# Autodesk Inventor assembly: Binary Clock
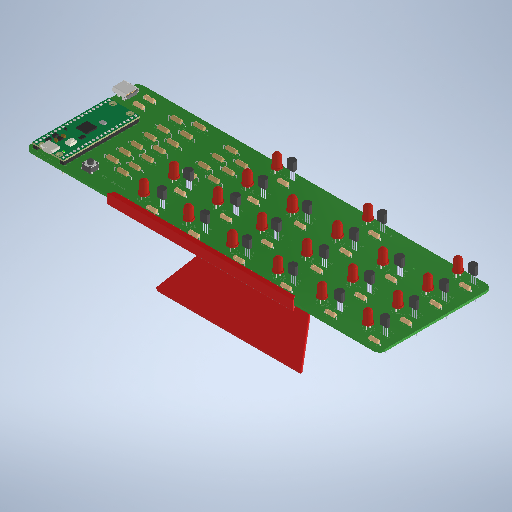
[picture p0: Inventor's stored thumbnail of the model, 512x512]
Saved by Autodesk Inventor 2025.3 (Build 293356000, 356)
## iProperties
Company: Kicad
Created: 2025-11-09
Part Number: Binary Clock
Description: KiCad electronic assembly
Document SubType Name: Assembly
Designer: User
Authority: Unknown
Sending System: KiCad to STEP converter
Preprocessor: Open CASCADE STEP processor 7.9
Title: Binary Clock.step
Author: Pcbnew
## Documents named in this file (11)
- C:\Users\User\Documents\KiCad\Binary Clock\Binary Clock\Binary Clock\Binary Clock\Binary Clock.iam
- C:\Users\User\Documents\KiCad\Binary Clock\Binary Clock\Binary Clock\Binary Clock\LED_D5.0mm.ipt
- C:\Users\User\Documents\KiCad\Binary Clock\Binary Clock\Binary Clock\Binary Clock\R_Axial_DIN0207_L6.3mm_D2.5mm_P7.62mm_Horizontal.ipt
- C:\Users\User\Documents\KiCad\Binary Clock\Binary Clock\Binary Clock\Binary Clock\RaspberryPi_Pico_H.iam
- C:\Users\User\Documents\KiCad\Binary Clock\Binary Clock\Binary Clock\Binary Clock\Binary Clock_silkscreen.ipt
- C:\Users\User\Documents\KiCad\Binary Clock\Binary Clock\Binary Clock\Binary Clock\Binary Clock_PCB.ipt
- C:\Users\User\3D\PC Case\Part14.ipt
- C:\Users\User\Documents\KiCad\Binary Clock\Binary Clock\Binary Clock\Binary Clock\R1.ipt
- C:\Users\User\Documents\KiCad\Binary Clock\Binary Clock\Binary Clock\Binary Clock\Same_Sky_TS02-66-70-BK-160-LCR-D.ipt
- C:\Users\User\Documents\KiCad\Binary Clock\Binary Clock\Binary Clock\Binary Clock\usb4085-gf-a.iam
- C:\Users\User\Downloads\BC547BBU\BC547BBU\BC547BBU.iam
## Components (88 placed, 50 different names)
1. 1
2. 2
3. 3
4. 4
5. 5
6. 6
7. 7
8. 8
9. 9
10. 10
11. 11
12. 12
13. 13
14. 14
15. 15
16. 16
17. 17
18. 18
19. 19
20. 20
21. 21
22. 22
23. 23
24. 24
25. 25
26. 26
27. 27
28. 28
29. 29
30. 30
31. 31
32. 32
33. 33
34. 34
35. 35
36. 36
37. 39 [sub-assembly]
38. 40
39. 41
40. 42
41. 43
42. 44
43. 45
44. 46
45. 47 — Flush:1, Mate:1, Mate:2, Mate:3, Mate:4, Mate:5, Mate:6, Mate:7, Mate:8, Mate:9, Mate:10, Mate:11, Mate:12, Mate:13, Mate:14, Mate:15, Mate:16, Mate:17, Mate:18, Mate:19, Mate:20, Mate:21, Mate:22, Mate:23, Mate:24, Mate:25, Mate:26, Mate:27, Mate:28, Mate:29, Mate:30, Mate:31, Mate:32, Mate:33, Mate:34, Mate:35, Mate:36, Mate:37, Mate:38, Mate:39, Mate:40, Mate:41, Mate:42
46. Part14:1 — Flush:1
47. R1:1 — Mate:2
48. R1:2 — Mate:1
49. R1:4 — Mate:3
50. R1:5 — Mate:6
51. R1:6 — Mate:4
52. R1:7 — Mate:12
53. R1:8 — Mate:8
54. R1:9 — Mate:7
55. R1:10 — Mate:5
56. R1:11 — Mate:15
57. R1:12 — Mate:14
58. R1:13 — Mate:9
59. R1:14 — Mate:11
60. R1:15 — Mate:18
61. R1:18 — Mate:17
62. R1:20 — Mate:20
63. R1:21 — Mate:13
64. R1:22 — Mate:19
65. R1:24 — Mate:16
66. R1:25 — Mate:10
67. Same_Sky_TS02-66-70-BK-160-LCR-D:1 — Mate:21
68. usb4085-gf-a:1 [sub-assembly] — Mate:22
69. BC547BBU:1 [sub-assembly] — Mate:23
70. BC547BBU:2 [sub-assembly] — Mate:24
71. BC547BBU:3 [sub-assembly] — Mate:25
72. BC547BBU:4 [sub-assembly] — Mate:26
73. BC547BBU:5 [sub-assembly] — Mate:33
74. BC547BBU:6 [sub-assembly] — Mate:27
75. BC547BBU:7 [sub-assembly] — Mate:28
76. BC547BBU:8 [sub-assembly] — Mate:32
77. BC547BBU:9 [sub-assembly] — Mate:31
78. BC547BBU:10 [sub-assembly] — Mate:29
79. BC547BBU:11 [sub-assembly] — Mate:30
80. BC547BBU:12 [sub-assembly] — Mate:37
81. BC547BBU:13 [sub-assembly] — Mate:35
82. BC547BBU:14 [sub-assembly] — Mate:34
83. BC547BBU:15 [sub-assembly] — Mate:38
84. BC547BBU:16 [sub-assembly] — Mate:36
85. BC547BBU:17 [sub-assembly] — Mate:40
86. BC547BBU:18 [sub-assembly] — Mate:42
87. BC547BBU:19 [sub-assembly] — Mate:39
88. BC547BBU:20 [sub-assembly] — Mate:41
## Relationships (43: Mate 42, Flush 1)
- Flush:1: 47 ↔ Part14:1
- Mate:1: 47 ↔ R1:2
- Mate:2: 47 ↔ R1:1
- Mate:3: 47 ↔ R1:4
- Mate:4: 47 ↔ R1:6
- Mate:5: 47 ↔ R1:10
- Mate:6: 47 ↔ R1:5
- Mate:7: 47 ↔ R1:9
- Mate:8: 47 ↔ R1:8
- Mate:9: 47 ↔ R1:13
- Mate:10: 47 ↔ R1:25
- Mate:11: 47 ↔ R1:14
- Mate:12: 47 ↔ R1:7
- Mate:13: 47 ↔ R1:21
- Mate:14: 47 ↔ R1:12
- Mate:15: 47 ↔ R1:11
- Mate:16: 47 ↔ R1:24
- Mate:17: 47 ↔ R1:18
- Mate:18: 47 ↔ R1:15
- Mate:19: 47 ↔ R1:22
- Mate:20: 47 ↔ R1:20
- Mate:21: 47 ↔ Same_Sky_TS02-66-70-BK-160-LCR-D:1
- Mate:22 (0.05 mm): 47 ↔ usb4085-gf-a:1
- Mate:23 (6 mm): 47 ↔ BC547BBU:1
- Mate:24 (6 mm): 47 ↔ BC547BBU:2
- Mate:25 (6 mm): 47 ↔ BC547BBU:3
- Mate:26 (6 mm): 47 ↔ BC547BBU:4
- Mate:27 (6 mm): 47 ↔ BC547BBU:6
- Mate:28 (6 mm): 47 ↔ BC547BBU:7
- Mate:29 (6 mm): 47 ↔ BC547BBU:10
- Mate:30 (6 mm): 47 ↔ BC547BBU:11
- Mate:31 (6 mm): 47 ↔ BC547BBU:9
- Mate:32 (6 mm): 47 ↔ BC547BBU:8
- Mate:33 (6 mm): 47 ↔ BC547BBU:5
- Mate:34 (6 mm): 47 ↔ BC547BBU:14
- Mate:35 (6 mm): 47 ↔ BC547BBU:13
- Mate:36 (6 mm): 47 ↔ BC547BBU:16
- Mate:37 (6 mm): 47 ↔ BC547BBU:12
- Mate:38 (6 mm): 47 ↔ BC547BBU:15
- Mate:39 (6 mm): 47 ↔ BC547BBU:19
- Mate:40 (6 mm): 47 ↔ BC547BBU:17
- Mate:41 (6 mm): 47 ↔ BC547BBU:20
- Mate:42 (6 mm): 47 ↔ BC547BBU:18
